# Autodesk Inventor assembly: CompBot 2019
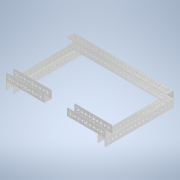
[picture p0: Inventor's stored thumbnail of the model, 180x180]
Saved by Autodesk Inventor 2020.1 (Build 241239000, 239)
## iProperties
Created: 2019-10-11
Part Number: CompBot 2019
Document SubType Name: Assembly
Designer: alpha
Author: alpha
## Documents named in this file (4)
- B:\Documents\GitHub\AO_Robotics\CAD\Projects\Joshua Schmidt\CompBot 2019.iam
- B:\Documents\GitHub\AO_Robotics\CAD\Parts Kits\FTC Tetrix KOP Organized (7-24-19)\Frame Hardware\Tetrix_39069.ipt
- B:\Documents\GitHub\AO_Robotics\CAD\Parts Kits\FTC Tetrix KOP Organized (7-24-19)\Frame Hardware\Tetrix_39068.ipt
- B:\Documents\GitHub\AO_Robotics\CAD\Parts Kits\FTC Tetrix KOP Organized (7-24-19)\Frame Hardware\Tetrix_39067.ipt
## Components (5 placed, 3 different names)
1. Tetrix_39069:1 — Mate:1, Mate:2, Rotational:1, Flush:1, Rotational:2, Flush:2
2. Tetrix_39068:1 — Rotational:1, Flush:1, Rotational:4, Flush:4
3. Tetrix_39068:2 — Rotational:2, Flush:2, Rotational:3, Flush:3
4. Tetrix_39067:1 — Rotational:3, Flush:3
5. Tetrix_39067:2 — Rotational:4, Flush:4
## Relationships (10: RevoluteJoint 4, Flush 4, Mate 2)
- Mate:1: Tetrix_39069:1
- Mate:2: Tetrix_39069:1
- Rotational:1 [RevoluteJoint]: Tetrix_39069:1 ↔ Tetrix_39068:1
- Flush:1: Tetrix_39069:1 ↔ Tetrix_39068:1
- Rotational:2 [RevoluteJoint]: Tetrix_39069:1 ↔ Tetrix_39068:2
- Flush:2: Tetrix_39069:1 ↔ Tetrix_39068:2
- Rotational:3 [RevoluteJoint]: Tetrix_39068:2 ↔ Tetrix_39067:1
- Flush:3: Tetrix_39068:2 ↔ Tetrix_39067:1
- Rotational:4 [RevoluteJoint]: Tetrix_39068:1 ↔ Tetrix_39067:2
- Flush:4: Tetrix_39068:1 ↔ Tetrix_39067:2
